# Autodesk Inventor assembly: Gotowy
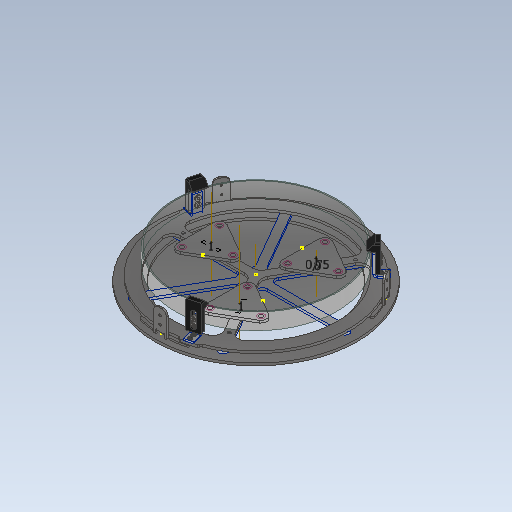
[picture p0: Inventor's stored thumbnail of the model, 512x512]
Saved by Autodesk Inventor 2020 (Build 240168000, 168)
## iProperties
Created: 2019-05-30
Part Number: Gotowy
Material: Ogólny
Document SubType Name: Assembly
Designer: barto
Author: barto
## Documents named in this file (21)
- C:\Users\Hesekiel\Desktop\Equatorial-Mount-MUM\Mechanika\Teleskop\Gotowy.iam
- C:\Users\Hesekiel\Desktop\Equatorial-Mount-MUM\Mechanika\Teleskop\RingPrimaryMirror.ipt
- C:\Users\Hesekiel\Desktop\Equatorial-Mount-MUM\Mechanika\Teleskop\NowyKatownik.ipt
- C:\Users\Hesekiel\Desktop\Equatorial-Mount-MUM\Mechanika\Teleskop\Połączenie gwintowe1.iam
- C:\Users\Hesekiel\Desktop\Equatorial-Mount-MUM\Mechanika\Teleskop\Połączenie gwintowe2.iam
- C:\Users\Hesekiel\Desktop\Equatorial-Mount-MUM\Mechanika\Teleskop\SpiderPrimaryMirror.ipt
- C:\Users\Hesekiel\Desktop\Equatorial-Mount-MUM\Mechanika\Teleskop\Połączenie gwintowe3.iam
- C:\Users\Hesekiel\Desktop\Equatorial-Mount-MUM\Mechanika\Teleskop\Połączenie gwintowe4.iam
- C:\Users\Hesekiel\Desktop\Equatorial-Mount-MUM\Mechanika\Teleskop\PrimaryMirror.ipt
- C:\Users\Hesekiel\Desktop\Equatorial-Mount-MUM\Mechanika\Teleskop\Połączenie gwintowe5.iam
- C:\Users\Hesekiel\Desktop\Equatorial-Mount-MUM\Mechanika\Teleskop\BearingBall.ipt
- C:\Users\Hesekiel\Desktop\Equatorial-Mount-MUM\Mechanika\Teleskop\HandlePrimaryMirror.ipt
- C:\Users\Hesekiel\Desktop\Equatorial-Mount-MUM\Mechanika\Teleskop\GumoweTrzymadlo.ipt
- C:\Users\Hesekiel\Desktop\Equatorial-Mount-MUM\Mechanika\Teleskop\Mirror.ipt
- C:\Users\Hesekiel\Desktop\Equatorial-Mount-MUM\Mechanika\Teleskop\Część4.ipt
- C:\Users\Hesekiel\Desktop\Equatorial-Mount-MUM\Mechanika\Teleskop\S-M3-0 ZI.ipt
- C:\Users\Hesekiel\Desktop\Equatorial-Mount-MUM\Mechanika\Teleskop\Trzymacz.ipt
- C:\Users\Hesekiel\Desktop\Equatorial-Mount-MUM\Mechanika\Teleskop\Połączenie gwintowe8.iam
- C:\Users\Hesekiel\Desktop\Equatorial-Mount-MUM\Mechanika\Teleskop\Połączenie gwintowe9.iam
- C:\Users\Hesekiel\Desktop\Equatorial-Mount-MUM\Mechanika\Teleskop\Połączenie gwintowe12.iam
- C:\Users\Hesekiel\Desktop\Equatorial-Mount-MUM\Mechanika\Teleskop\Połączenie gwintowe14.iam
## Components (61 placed, 12 different names)
1. RingPrimaryMirror:1 — Zestawiające:1, Zestawiające:2, Zestawiające:3, Zestawiające:4, Zestawiające:5, Zestawiające:6, Zestawiające:7, Zestawiające:8, Zestawiające:9, Zestawiające:10, Zestawiające:11, Zestawiające:13, Zestawiające:14
2. SpiderPrimaryMirror:1 — Zestawiające:8, Zestawiające:9, Zestawiające:10, Zestawiające:12, Zestawiające:15, Zestawiające:16, Zestawiające:17, Zestawiające:18
3. PrimaryMirror:1 — Zestawiające:15, Zestawiające:16, Zestawiające:17, Zestawiające:19, Zestawiające:20, Zestawiające:21, Zestawiające:22, Kątowe:1, Zestawiające:27, Zestawiające:28, Zestawiające:29, Zestawiające:30
4. Mirror:1 — Zestawiające:26, Zestawiające:27, Zestawiające:40
5. NowyKatownik:1 — Zestawiające:1, Zestawiające:2, Zestawiające:3
6. NowyKatownik:2
7. NowyKatownik:3
8. Połączenie gwintowe:2 [sub-assembly] — Zestawiające:6, Zestawiające:7
9. Połączenie gwintowe:1 [sub-assembly] — Zestawiające:4, Zestawiające:5
10. Połączenie gwintowe:3 [sub-assembly]
11. Połączenie gwintowe:4 [sub-assembly]
12. Połączenie gwintowe:5 [sub-assembly]
13. Połączenie gwintowe:6 [sub-assembly]
14. Połączenie gwintowe:7 [sub-assembly] — Zestawiające:11, Zestawiające:12
15. Połączenie gwintowe:8 [sub-assembly]
16. Połączenie gwintowe:9 [sub-assembly]
17. Połączenie gwintowe:10 [sub-assembly] — Zestawiające:13, Zestawiające:14
18. Połączenie gwintowe:11 [sub-assembly]
19. Połączenie gwintowe:12 [sub-assembly]
20. Połączenie gwintowe:13 [sub-assembly] — Zestawiające:18, Zestawiające:19
21. Połączenie gwintowe:14 [sub-assembly]
22. Połączenie gwintowe:15 [sub-assembly]
23. BearingBall:1 — Zestawiające:20, Zestawiające:21
24. BearingBall:2 — Zestawiające:23
25. BearingBall:3
26. HandlePrimaryMirror:1 — Zestawiające:22, Zestawiające:23
27. HandlePrimaryMirror:2 — Kątowe:1, Zestawiające:24, Zestawiające:25, Zestawiające:26
28. HandlePrimaryMirror:3
29. Część4:1 — Zestawiające:28, Zestawiające:29, Zestawiające:30, Zestawiające:31, Zestawiające:32, Zestawiające:33, Zestawiające:34, Zestawiające:39, Równoległe:1, Zestawiające:51, Zestawiające:52, Zestawiające:53, Zestawiające:54
30. PEM Nakrętki samozaciskowe S,SS,CLS,CLSS - Metryczny S-M3-0 ZI:1 — Zestawiające:31, Zestawiające:32, Zestawiające:48
31. PEM Nakrętki samozaciskowe S,SS,CLS,CLSS - Metryczny S-M3-0 ZI:2 — Zestawiające:33, Zestawiające:34, Zestawiające:46
32. Część4:2
33. PEM Nakrętki samozaciskowe S,SS,CLS,CLSS - Metryczny S-M3-0 ZI:3
34. PEM Nakrętki samozaciskowe S,SS,CLS,CLSS - Metryczny S-M3-0 ZI:4
35. Część4:3
36. PEM Nakrętki samozaciskowe S,SS,CLS,CLSS - Metryczny S-M3-0 ZI:5
37. PEM Nakrętki samozaciskowe S,SS,CLS,CLSS - Metryczny S-M3-0 ZI:6
38. Trzymacz:1 — Zestawiające:39, Równoległe:1, Zestawiające:40, Zestawiające:45, Zestawiające:47
39. Trzymacz:2
40. Trzymacz:3
41. Połączenie gwintowe:21 [sub-assembly] — Zestawiające:51, Zestawiające:52
42. Połączenie gwintowe:22 [sub-assembly] — Zestawiające:53, Zestawiające:54
43. Połączenie gwintowe:18 [sub-assembly] — Zestawiające:45, Zestawiające:46
44. Połączenie gwintowe:19 [sub-assembly] — Zestawiające:47, Zestawiające:48
45. Połączenie gwintowe:23 [sub-assembly]
46. Połączenie gwintowe:24 [sub-assembly]
47. Połączenie gwintowe:25 [sub-assembly]
48. Połączenie gwintowe:26 [sub-assembly]
49. Połączenie gwintowe:27 [sub-assembly]
50. Połączenie gwintowe:28 [sub-assembly]
51. Połączenie gwintowe:29 [sub-assembly]
52. Połączenie gwintowe:30 [sub-assembly]
53. GumoweTrzymadlo:1 — Zestawiające:24, Zestawiające:25
54. GumoweTrzymadlo:2
55. GumoweTrzymadlo:3
56. GumoweTrzymadlo:4
57. GumoweTrzymadlo:5
58. GumoweTrzymadlo:6
59. GumoweTrzymadlo:7
60. GumoweTrzymadlo:8
61. GumoweTrzymadlo:9
## Component patterns: (3 elements, first: NowyKatownik:1), (3 elements, first: Połączenie gwintowe:2 + Połączenie gwintowe:1), (3 elements, first: Połączenie gwintowe:7), (3 elements, first: Połączenie gwintowe:10), (3 elements, first: Połączenie gwintowe:13), (3 elements, first: BearingBall:1), (3 elements, first: HandlePrimaryMirror:1), (3 elements), (3 elements, first: Część4:1 + PEM Nakrętki samozaciskowe S,SS,CLS,CLSS - Metryczny S-M3-0 ZI:1 + PEM Nakrętki samozaciskowe S,SS,CLS,CLSS - Metryczny S-M3-0 ZI:2), (3 elements, first: Trzymacz:1), (3 elements, first: Połączenie gwintowe:21 + Połączenie gwintowe:22 + Połączenie gwintowe:18 + Połączenie gwintowe:19), (3 elements, first: GumoweTrzymadlo:1), Szyk komponentów 8:2 (3 elements), Szyk komponentów 8:3 (3 elements)
## Relationships (46: Mate 44, Angle 1, Flush 1)
- Zestawiające:1 [Mate] (0.3 mm): RingPrimaryMirror:1 ↔ NowyKatownik:1
- Zestawiające:2 [Mate]: RingPrimaryMirror:1 ↔ NowyKatownik:1
- Zestawiające:3 [Mate]: RingPrimaryMirror:1 ↔ NowyKatownik:1
- Zestawiające:4 [Mate]: RingPrimaryMirror:1 ↔ Połączenie gwintowe:1
- Zestawiające:5 [Mate]: RingPrimaryMirror:1 ↔ Połączenie gwintowe:1
- Zestawiające:6 [Mate]: RingPrimaryMirror:1 ↔ Połączenie gwintowe:2
- Zestawiające:7 [Mate]: RingPrimaryMirror:1 ↔ Połączenie gwintowe:2
- Zestawiające:8 [Mate]: RingPrimaryMirror:1 ↔ SpiderPrimaryMirror:1
- Zestawiające:9 [Mate]: RingPrimaryMirror:1 ↔ SpiderPrimaryMirror:1
- Zestawiające:10 [Mate]: RingPrimaryMirror:1 ↔ SpiderPrimaryMirror:1
- Zestawiające:11 [Mate]: RingPrimaryMirror:1 ↔ Połączenie gwintowe:7
- Zestawiające:12 [Mate]: SpiderPrimaryMirror:1 ↔ Połączenie gwintowe:7
- Zestawiające:13 [Mate] (2 mm): RingPrimaryMirror:1 ↔ Połączenie gwintowe:10
- Zestawiające:14 [Mate]: RingPrimaryMirror:1 ↔ Połączenie gwintowe:10
- Zestawiające:15 [Mate]: SpiderPrimaryMirror:1 ↔ PrimaryMirror:1
- Zestawiające:16 [Mate]: SpiderPrimaryMirror:1 ↔ PrimaryMirror:1
- Zestawiające:17 [Mate]: SpiderPrimaryMirror:1 ↔ PrimaryMirror:1
- Zestawiające:18 [Mate]: SpiderPrimaryMirror:1 ↔ Połączenie gwintowe:13
- Zestawiające:19 [Mate]: PrimaryMirror:1 ↔ Połączenie gwintowe:13
- Zestawiające:20 [Mate]: PrimaryMirror:1 ↔ BearingBall:1
- Zestawiające:21 [Mate] (1.965 mm): PrimaryMirror:1 ↔ BearingBall:1
- Zestawiające:22 [Mate]: PrimaryMirror:1 ↔ HandlePrimaryMirror:1
- Zestawiające:23 [Mate] (1.965 mm): BearingBall:2 ↔ HandlePrimaryMirror:1
- Kątowe:1 [Angle] (90 deg): PrimaryMirror:1 ↔ HandlePrimaryMirror:2
- Zestawiające:24 [Mate]: HandlePrimaryMirror:2 ↔ GumoweTrzymadlo:1
- Zestawiające:25 [Mate]: HandlePrimaryMirror:2 ↔ GumoweTrzymadlo:1
- Zestawiające:26 [Mate] (4 mm): Mirror:1 ↔ HandlePrimaryMirror:2
- Zestawiające:27 [Mate]: PrimaryMirror:1 ↔ Mirror:1
- Zestawiające:28 [Mate]: PrimaryMirror:1 ↔ Część4:1
- Zestawiające:29 [Mate]: PrimaryMirror:1 ↔ Część4:1
- Zestawiające:30 [Mate]: PrimaryMirror:1 ↔ Część4:1
- Zestawiające:31 [Mate]: Część4:1 ↔ PEM Nakrętki samozaciskowe S,SS,CLS,CLSS - Metryczny S-M3-0 ZI:1
- Zestawiające:32 [Mate]: Część4:1 ↔ PEM Nakrętki samozaciskowe S,SS,CLS,CLSS - Metryczny S-M3-0 ZI:1
- Zestawiające:33 [Mate]: Część4:1 ↔ PEM Nakrętki samozaciskowe S,SS,CLS,CLSS - Metryczny S-M3-0 ZI:2
- Zestawiające:34 [Mate]: Część4:1 ↔ PEM Nakrętki samozaciskowe S,SS,CLS,CLSS - Metryczny S-M3-0 ZI:2
- Zestawiające:39 [Mate]: Część4:1 ↔ Trzymacz:1
- Równoległe:1 [Flush] (3 mm): Część4:1 ↔ Trzymacz:1
- Zestawiające:40 [Mate] (-1 mm): Mirror:1 ↔ Trzymacz:1
- Zestawiające:45 [Mate]: Trzymacz:1 ↔ Połączenie gwintowe:18
- Zestawiające:46 [Mate]: PEM Nakrętki samozaciskowe S,SS,CLS,CLSS - Metryczny S-M3-0 ZI:2 ↔ Połączenie gwintowe:18
- Zestawiające:47 [Mate]: Trzymacz:1 ↔ Połączenie gwintowe:19
- Zestawiające:48 [Mate]: PEM Nakrętki samozaciskowe S,SS,CLS,CLSS - Metryczny S-M3-0 ZI:1 ↔ Połączenie gwintowe:19
- Zestawiające:51 [Mate]: Część4:1 ↔ Połączenie gwintowe:21
- Zestawiające:52 [Mate]: Część4:1 ↔ Połączenie gwintowe:21
- Zestawiające:53 [Mate]: Część4:1 ↔ Połączenie gwintowe:22
- Zestawiające:54 [Mate]: Część4:1 ↔ Połączenie gwintowe:22
